# Autodesk Inventor assembly: FE-00035-01
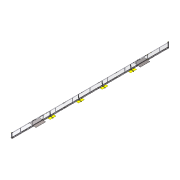
[picture p0: Inventor's stored thumbnail of the model, 180x180]
Saved by Autodesk Inventor 2012 (Build 160160000, 160)
## iProperties
Created: 2010-11-28
Part Number: FE-00035-01
Document SubType Name: Assembly
Designer: dfoster
Stock Number: Side Border Sub-Assembly
Title: Side Border Sub-Assembly
Author: dfoster
## Documents named in this file (13)
- C:\Data Folder\FRC 2012 Field\Components\FE-00035-01.iam
- C:\Data Folder\FRC 2012 Field\Components\FE-00024.iam
- C:\Data Folder\FRC 2012 Field\Components\FE-00023.iam
- C:\Data Folder\FRC 2012 Field\Components\FE-00022.iam
- C:\Data Folder\FRC 2012 Field\Components\FE-00013.iam
- C:\Data Folder\FRC 2012 Field\Components\FE-00029.iam
- C:\Data Folder\FRC 2012 Field\Components\FE-00014.iam
- C:\Data Folder\FRC 2012 Field\Components\FE-00015.ipt
- C:\Data Folder\FRC 2012 Field\Components\FE-00003.iam
- C:\Data Folder\FRC 2012 Field\Components\FE-00008.ipt
- C:\Data Folder\FRC 2012 Field\Components\FE-00009.ipt
- C:\Data Folder\FRC 2012 Field\Components\FE-00010.ipt
- C:\Data Folder\FRC 2012 Field\Components\FE-00017.iam
## Components (33 placed, 12 different names)
1. FE-00003:1 [sub-assembly] — Mate:35, Flush:22, Angle:2
2. FE-00003:2 [sub-assembly] — Mate:36, Flush:23, Angle:3
3. FE-00014:1 [sub-assembly] — Mate:32, Mate:33, Mate:34, Flush:21
4. FE-00014:2 [sub-assembly] — Mate:29, Mate:30, Mate:31, Flush:20
5. FE-00015:1 — Mate:17, Mate:21, Mate:22
6. FE-00015:2 — Mate:18, Mate:23, Mate:24
7. FE-00015:3 — Mate:19, Mate:25, Mate:26
8. FE-00015:4 — Mate:20, Mate:27, Mate:28
9. FE-00013:1 [sub-assembly] — Mate:15, Mate:16, Flush:17, Angle:1, Mate:20, Mate:27, Mate:28
10. FE-00013:2 [sub-assembly] — Mate:13, Mate:14, Flush:17, Flush:18, Mate:19, Mate:25, Mate:26
11. FE-00013:3 [sub-assembly] — Mate:11, Mate:12, Flush:18, Flush:19, Mate:18, Mate:23, Mate:24
12. FE-00013:4 [sub-assembly] — Mate:9, Mate:10, Flush:19, Mate:17, Mate:21, Mate:22
13. FE-00029:2 [sub-assembly] — Flush:13, Flush:14, Flush:15, Flush:16, Mate:7, Mate:8, Mate:29, Mate:30, Mate:31, Flush:20, Mate:56, Mate:58, Flush:32, Mate:70
14. FE-00029:1 [sub-assembly] — Flush:1, Flush:2, Flush:3, Flush:4, Mate:1, Mate:2, Mate:32, Mate:33, Mate:34, Flush:21, Mate:41, Mate:42, Mate:44
15. FE-00022:5 [sub-assembly] — Flush:11, Flush:12, Flush:13, Flush:14, Mate:6, Mate:7, Mate:9, Mate:10, Mate:54, Mate:55, Flush:31
16. FE-00022:4 [sub-assembly] — Flush:7, Flush:8, Flush:9, Flush:10, Mate:4, Mate:5, Mate:50, Mate:51, Flush:29, Mate:74, Mate:75, Mate:76
17. FE-00022:3 [sub-assembly] — Flush:5, Flush:6, Flush:7, Flush:8, Mate:3, Mate:4, Mate:13, Mate:14, Mate:48, Mate:49, Flush:28
18. FE-00022:1 [sub-assembly] — Flush:9, Flush:10, Flush:11, Flush:12, Mate:5, Mate:6, Mate:11, Mate:12, Flush:30, Mate:68, Mate:69
19. FE-00024:1 [sub-assembly] — Flush:15, Flush:16, Mate:8, Mate:35, Flush:22, Angle:2, Flush:33, Mate:71, Mate:72, Mate:73
20. FE-00023:1 [sub-assembly] — Flush:1, Flush:2, Mate:1, Mate:36, Flush:23, Angle:3, Flush:24, Flush:25, Mate:63, Mate:64, Mate:65, Mate:66
21. FE-00022:2 [sub-assembly] — Flush:3, Flush:4, Flush:5, Flush:6, Mate:2, Mate:3, Mate:15, Mate:16, Angle:1, Mate:43, Flush:26, Mate:46, Mate:47, Flush:27
22. FE-00009:1 — Flush:25, Mate:65, Mate:66, Mate:67
23. FE-00010:1 — Flush:30, Mate:68, Mate:69
24. FE-00009:2 — Flush:32, Mate:70, Mate:71
25. FE-00008:2 — Flush:24, Mate:63, Mate:64
26. FE-00008:1 — Flush:33, Mate:72, Mate:73
27. FE-00010:2 — Mate:46, Mate:47, Flush:27
28. FE-00017:2 [sub-assembly] — Mate:56, Mate:57, Mate:58
29. FE-00017:1 [sub-assembly] — Mate:41, Mate:42, Mate:67
30. FE-00009:3 — Mate:43, Flush:26, Mate:44
31. FE-00010:3 — Mate:48, Mate:49, Flush:28
32. FE-00010:4 — Mate:50, Mate:51, Flush:29
33. FE-00009:4 — Mate:54, Mate:55, Flush:31, Mate:57
## Relationships (101: Mate 65, Flush 33, Angle 3)
- Flush:1: FE-00029:1 ↔ FE-00023:1
- Flush:2: FE-00029:1 ↔ FE-00023:1
- Flush:3: FE-00029:1 ↔ FE-00022:2
- Flush:4: FE-00029:1 ↔ FE-00022:2
- Flush:5: FE-00022:3 ↔ FE-00022:2
- Flush:6: FE-00022:3 ↔ FE-00022:2
- Flush:7: FE-00022:4 ↔ FE-00022:3
- Flush:8: FE-00022:4 ↔ FE-00022:3
- Flush:9: FE-00022:4 ↔ FE-00022:1
- Flush:10: FE-00022:4 ↔ FE-00022:1
- Flush:11: FE-00022:5 ↔ FE-00022:1
- Flush:12: FE-00022:5 ↔ FE-00022:1
- Flush:13: FE-00029:2 ↔ FE-00022:5
- Flush:14: FE-00029:2 ↔ FE-00022:5
- Flush:15: FE-00029:2 ↔ FE-00024:1
- Flush:16: FE-00029:2 ↔ FE-00024:1
- Mate:1: FE-00029:1 ↔ FE-00023:1
- Mate:2: FE-00029:1 ↔ FE-00022:2
- Mate:3: FE-00022:3 ↔ FE-00022:2
- Mate:4: FE-00022:4 ↔ FE-00022:3
- Mate:5: FE-00022:4 ↔ FE-00022:1
- Mate:6: FE-00022:5 ↔ FE-00022:1
- Mate:7: FE-00029:2 ↔ FE-00022:5
- Mate:8: FE-00029:2 ↔ FE-00024:1
- Mate:9: FE-00013:4 ↔ FE-00022:5
- Mate:10: FE-00013:4 ↔ FE-00022:5
- Mate:11: FE-00013:3 ↔ FE-00022:1
- Mate:12: FE-00013:3 ↔ FE-00022:1
- Mate:13: FE-00013:2 ↔ FE-00022:3
- Mate:14: FE-00013:2 ↔ FE-00022:3
- Mate:15: FE-00013:1 ↔ FE-00022:2
- Mate:16: FE-00013:1 ↔ FE-00022:2
- Flush:17: FE-00013:1 ↔ FE-00013:2
- Flush:18: FE-00013:2 ↔ FE-00013:3
- Flush:19: FE-00013:3 ↔ FE-00013:4
- Angle:1 (0 deg): FE-00013:1 ↔ FE-00022:2
- Mate:17: FE-00015:1 ↔ FE-00013:4
- Mate:18: FE-00015:2 ↔ FE-00013:3
- Mate:19: FE-00015:3 ↔ FE-00013:2
- Mate:20: FE-00015:4 ↔ FE-00013:1
- Mate:21 (4.7752 mm): FE-00015:1 ↔ FE-00013:4
- Mate:22: FE-00015:1 ↔ FE-00013:4
- Mate:23 (4.7752 mm): FE-00015:2 ↔ FE-00013:3
- Mate:24: FE-00015:2 ↔ FE-00013:3
- Mate:25 (4.7752 mm): FE-00015:3 ↔ FE-00013:2
- Mate:26: FE-00015:3 ↔ FE-00013:2
- Mate:27 (4.7752 mm): FE-00015:4 ↔ FE-00013:1
- Mate:28: FE-00015:4 ↔ FE-00013:1
- Mate:29: FE-00014:2 ↔ FE-00029:2
- Mate:30: FE-00014:2 ↔ FE-00029:2
- Mate:31: FE-00014:2 ↔ FE-00029:2
- Flush:20 (38.1 mm): FE-00014:2 ↔ FE-00029:2
- Mate:32: FE-00014:1 ↔ FE-00029:1
- Mate:33: FE-00014:1 ↔ FE-00029:1
- Mate:34: FE-00014:1 ↔ FE-00029:1
- Flush:21 (38.1 mm): FE-00014:1 ↔ FE-00029:1
- Mate:35: FE-00003:1 ↔ FE-00024:1
- Flush:22: FE-00003:1 ↔ FE-00024:1
- Angle:2 (180 deg): FE-00003:1 ↔ FE-00024:1
- Mate:36: FE-00003:2 ↔ FE-00023:1
- Flush:23: FE-00003:2 ↔ FE-00023:1
- Angle:3 (0 deg): FE-00003:2 ↔ FE-00023:1
- Flush:24: FE-00023:1 ↔ FE-00008:2
- Flush:25: FE-00023:1 ↔ FE-00009:1
- Mate:41: FE-00029:1 ↔ FE-00017:1
- Mate:42: FE-00029:1 ↔ FE-00017:1
- Mate:43: FE-00022:2 ↔ FE-00009:3
- Flush:26: FE-00022:2 ↔ FE-00009:3
- Mate:44: FE-00029:1 ↔ FE-00009:3
- Mate:46: FE-00022:2 ↔ FE-00010:2
- Mate:47: FE-00022:2 ↔ FE-00010:2
- Flush:27: FE-00022:2 ↔ FE-00010:2
- Mate:48: FE-00022:3 ↔ FE-00010:3
- Mate:49: FE-00022:3 ↔ FE-00010:3
- Flush:28: FE-00022:3 ↔ FE-00010:3
- Mate:50: FE-00022:4 ↔ FE-00010:4
- Mate:51: FE-00022:4 ↔ FE-00010:4
- Flush:29: FE-00022:4 ↔ FE-00010:4
- Flush:30: FE-00022:1 ↔ FE-00010:1
- Mate:54: FE-00022:5 ↔ FE-00009:4
- Mate:55: FE-00022:5 ↔ FE-00009:4
- Flush:31: FE-00022:5 ↔ FE-00009:4
- Mate:56: FE-00029:2 ↔ FE-00017:2
- Mate:57 (35.56 mm): FE-00017:2 ↔ FE-00009:4
- Mate:58: FE-00029:2 ↔ FE-00017:2
- Flush:32: FE-00029:2 ↔ FE-00009:2
- Flush:33: FE-00024:1 ↔ FE-00008:1
- Mate:63: FE-00023:1 ↔ FE-00008:2
- Mate:64: FE-00023:1 ↔ FE-00008:2
- Mate:65: FE-00023:1 ↔ FE-00009:1
- Mate:66: FE-00023:1 ↔ FE-00009:1
- Mate:67 (35.56 mm): FE-00009:1 ↔ FE-00017:1
- Mate:68: FE-00022:1 ↔ FE-00010:1
- Mate:69: FE-00022:1 ↔ FE-00010:1
- Mate:70: FE-00029:2 ↔ FE-00009:2
- Mate:71: FE-00024:1 ↔ FE-00009:2
- Mate:72: FE-00024:1 ↔ FE-00008:1
- Mate:73: FE-00024:1 ↔ FE-00008:1
- Mate:74: FE-00022:4
- Mate:75: FE-00022:4
- Mate:76: FE-00022:4
